# Autodesk Inventor assembly: zlozenieTymRazemOdwrotniezUchwytem
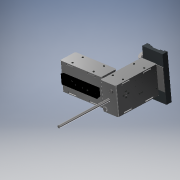
[picture p0: Inventor's stored thumbnail of the model, 180x180]
Saved by Autodesk Inventor 2019.4 (Build 234330000, 330)
## iProperties
Created: 2020-08-29
Part Number: zlozenieTymRazemOdwrotniezUchwytem
Document SubType Name: Assembly
Designer: estee
Author: estee
## Documents named in this file (16)
- F:\GitHub\MUMv2\Equatorial-Mount-MUM\Mechanika\Moduł obrotu RET Estera\projejt\projejt\NoweZlozenie\zlozenieTymRazemOdwrotniezUchwytem.iam
- F:\GitHub\MUMv2\Equatorial-Mount-MUM\Mechanika\Moduł obrotu RET Estera\projejt\projejt\NoweZlozenie\ObudowaNowa.iam
- F:\GitHub\MUMv2\Equatorial-Mount-MUM\Mechanika\Moduł obrotu RET Estera\projejt\projejt\NoweZlozenie\ObudowaNowa2.iam
- F:\GitHub\MUMv2\Equatorial-Mount-MUM\Mechanika\Moduł obrotu RET Estera\projejt\projejt\NoweZlozenie\ISO 4026 - M3 x 3 - ISO.ipt
- F:\GitHub\MUMv2\Equatorial-Mount-MUM\Mechanika\Moduł obrotu RET Estera\projejt\projejt\NoweZlozenie\trzymak.iam
- F:\GitHub\MUMv2\Equatorial-Mount-MUM\Mechanika\Moduł obrotu RET Estera\projejt\projejt\NoweZlozenie\dovetail.ipt
- F:\GitHub\MUMv2\Equatorial-Mount-MUM\Mechanika\Moduł obrotu RET Estera\projejt\projejt\NoweZlozenie\Połączenie gwintowe1.iam
- F:\GitHub\MUMv2\Equatorial-Mount-MUM\Mechanika\Moduł obrotu RET Estera\projejt\projejt\NoweZlozenie\Połączenie gwintowe2.iam
- F:\GitHub\MUMv2\Equatorial-Mount-MUM\Mechanika\Moduł obrotu RET Estera\projejt\projejt\NoweZlozenie\Połączenie gwintowe4.iam
- F:\GitHub\MUMv2\Equatorial-Mount-MUM\Mechanika\Moduł obrotu RET Estera\projejt\projejt\NoweZlozenie\Połączenie gwintowe5.iam
- F:\GitHub\MUMv2\Equatorial-Mount-MUM\Mechanika\Moduł obrotu RET Estera\projejt\projejt\NoweZlozenie\Połączenie gwintowe6.iam
- F:\GitHub\MUMv2\Equatorial-Mount-MUM\Mechanika\Moduł obrotu RET Estera\projejt\projejt\NoweZlozenie\Połączenie gwintowe7.iam
- F:\GitHub\MUMv2\Equatorial-Mount-MUM\Mechanika\Moduł obrotu RET Estera\projejt\projejt\NoweZlozenie\Połączenie gwintowe8.iam
- F:\GitHub\MUMv2\Equatorial-Mount-MUM\Mechanika\Moduł obrotu RET Estera\projejt\projejt\NoweZlozenie\Połączenie gwintowe9.iam
- F:\GitHub\MUMv2\Equatorial-Mount-MUM\Mechanika\Moduł obrotu RET Estera\projejt\projejt\NoweZlozenie\ISO 8676 - M10 x 1 x 20 - ISO.ipt
- F:\GitHub\MUMv2\Equatorial-Mount-MUM\Mechanika\Moduł obrotu RET Estera\projejt\projejt\NoweZlozenie\ISO 4035 - M10 - ISO.ipt
## Components (34 placed, 8 different names)
1. ObudowaNowa:1 [sub-assembly] — Angle:1, Tangent:1, Tangent:2, Tangent:3, Tangent:4, Mate:14, Mate:15, Zestawiające:16, Zestawiające:17, Zestawiające:18, Mate:35, Mate:36, Mate:38, Mate:39, Mate:40, Mate:42, Mate:43, Mate:44, Mate:45, Mate:46, Mate:47, Mate:48, Mate:49, Mate:50
2. ObudowaNowa2:1 [sub-assembly] — Angle:1, Mate:3, Mate:4, Mate:5, Mate:6, Mate:7, Mate:8, Angle:2, Tangent:5, Tangent:6, Mate:13, Mate:14, Mate:15, Mate:51, Mate:52, Mate:53, Mate:54, Mate:55, Mate:56, Mate:57, Mate:58, Mate:59, Mate:60, Mate:61, Mate:62, Mate:63, Mate:64, Mate:65, Mate:66
3. ISO 4026 M3 x 3:1 — Mate:7, Tangent:4
4. ISO 4026 M3 x 3:2 — Mate:5, Tangent:3
5. ISO 4026 M3 x 3:3 — Mate:3, Mate:6, Tangent:1
6. ISO 4026 M3 x 3:4 — Mate:4, Tangent:2
7. trzymak:1 [sub-assembly] — Mate:8, Angle:2, Mate:11, Mate:12, Mate:13
8. ISO 4026 M3 x 3:5 — Mate:11, Tangent:5
9. ISO 4026 M3 x 3:6 — Mate:12, Tangent:6
10. dovetail:1 — Zestawiające:16, Zestawiające:17, Zestawiające:18, Zestawiające:19, Zestawiające:20, Zestawiające:21, Zestawiające:22, Zestawiające:23, Zestawiające:24, Zestawiające:25, Zestawiające:26, Zestawiające:27, Zestawiające:28, Zestawiające:29, Zestawiające:30, Zestawiające:31, Zestawiające:32, Zestawiające:33, Zestawiające:34
11. Połączenie gwintowe:1 [sub-assembly] — Zestawiające:19, Zestawiające:20
12. Połączenie gwintowe:2 [sub-assembly] — Zestawiające:21, Zestawiające:22
13. Połączenie gwintowe:3 [sub-assembly] — Zestawiające:23, Zestawiające:24
14. Połączenie gwintowe:4 [sub-assembly] — Zestawiające:25, Zestawiające:26
15. Połączenie gwintowe:5 [sub-assembly] — Zestawiające:27, Zestawiające:28
16. Połączenie gwintowe:6 [sub-assembly] — Zestawiające:29, Zestawiające:30
17. Połączenie gwintowe:7 [sub-assembly] — Zestawiające:31, Zestawiające:32
18. Połączenie gwintowe:8 [sub-assembly] — Zestawiające:33, Zestawiające:34
19. ISO 8676 M10 x 1 x 20:1 — Mate:35, Mate:36, Mate:37
20. ISO 4035 M10:1 — Mate:37, Mate:38
21. ISO 8676 M10 x 1 x 20:2 — Mate:39, Mate:40, Mate:41
22. ISO 4035 M10:2 — Mate:41, Mate:42
23. ISO 4035 M10:3 — Mate:43, Mate:44
24. ISO 4035 M10:4 — Mate:45, Mate:46
25. ISO 8676 M10 x 1 x 20:3 — Mate:47, Mate:49
26. ISO 8676 M10 x 1 x 20:4 — Mate:48, Mate:50
27. ISO 4035 M10:5 — Mate:51, Mate:54
28. ISO 4035 M10:6 — Mate:55, Mate:56
29. ISO 4035 M10:7 — Mate:52, Mate:53
30. ISO 4035 M10:8 — Mate:57, Mate:58
31. ISO 8676 M10 x 1 x 20:5 — Mate:59, Mate:61
32. ISO 8676 M10 x 1 x 20:6 — Mate:60, Mate:62
33. ISO 8676 M10 x 1 x 20:7 — Mate:65, Mate:66
34. ISO 8676 M10 x 1 x 20:8 — Mate:63, Mate:64
## Relationships (70: Mate 62, Tangent 6, Angle 2)
- Angle:1 (0 deg): ObudowaNowa:1 ↔ ObudowaNowa2:1
- Mate:3: ObudowaNowa2:1 ↔ ISO 4026 M3 x 3:3
- Mate:4: ObudowaNowa2:1 ↔ ISO 4026 M3 x 3:4
- Mate:5: ObudowaNowa2:1 ↔ ISO 4026 M3 x 3:2
- Mate:6: ObudowaNowa2:1 ↔ ISO 4026 M3 x 3:3
- Tangent:1: ObudowaNowa:1 ↔ ISO 4026 M3 x 3:3
- Tangent:2: ObudowaNowa:1 ↔ ISO 4026 M3 x 3:4
- Tangent:3: ObudowaNowa:1 ↔ ISO 4026 M3 x 3:2
- Mate:7: ObudowaNowa2:1 ↔ ISO 4026 M3 x 3:1
- Tangent:4: ObudowaNowa:1 ↔ ISO 4026 M3 x 3:1
- Mate:8: ObudowaNowa2:1 ↔ trzymak:1
- Angle:2 (0 deg): ObudowaNowa2:1 ↔ trzymak:1
- Mate:11: trzymak:1 ↔ ISO 4026 M3 x 3:5
- Tangent:5: ObudowaNowa2:1 ↔ ISO 4026 M3 x 3:5
- Mate:12: trzymak:1 ↔ ISO 4026 M3 x 3:6
- Tangent:6: ObudowaNowa2:1 ↔ ISO 4026 M3 x 3:6
- Mate:13: ObudowaNowa2:1 ↔ trzymak:1
- Mate:14: ObudowaNowa:1 ↔ ObudowaNowa2:1
- Mate:15 (5 mm): ObudowaNowa:1 ↔ ObudowaNowa2:1
- Zestawiające:16 [Mate]: ObudowaNowa:1 ↔ dovetail:1
- Zestawiające:17 [Mate]: ObudowaNowa:1 ↔ dovetail:1
- Zestawiające:18 [Mate]: ObudowaNowa:1 ↔ dovetail:1
- Zestawiające:19 [Mate]: dovetail:1 ↔ Połączenie gwintowe:1
- Zestawiające:20 [Mate]: dovetail:1 ↔ Połączenie gwintowe:1
- Zestawiające:21 [Mate]: dovetail:1 ↔ Połączenie gwintowe:2
- Zestawiające:22 [Mate]: dovetail:1 ↔ Połączenie gwintowe:2
- Zestawiające:23 [Mate]: dovetail:1 ↔ Połączenie gwintowe:3
- Zestawiające:24 [Mate]: dovetail:1 ↔ Połączenie gwintowe:3
- Zestawiające:25 [Mate]: dovetail:1 ↔ Połączenie gwintowe:4
- Zestawiające:26 [Mate]: dovetail:1 ↔ Połączenie gwintowe:4
- Zestawiające:27 [Mate]: dovetail:1 ↔ Połączenie gwintowe:5
- Zestawiające:28 [Mate]: dovetail:1 ↔ Połączenie gwintowe:5
- Zestawiające:29 [Mate]: dovetail:1 ↔ Połączenie gwintowe:6
- Zestawiające:30 [Mate]: dovetail:1 ↔ Połączenie gwintowe:6
- Zestawiające:31 [Mate]: dovetail:1 ↔ Połączenie gwintowe:7
- Zestawiające:32 [Mate]: dovetail:1 ↔ Połączenie gwintowe:7
- Zestawiające:33 [Mate]: dovetail:1 ↔ Połączenie gwintowe:8
- Zestawiające:34 [Mate]: dovetail:1 ↔ Połączenie gwintowe:8
- Mate:35: ObudowaNowa:1 ↔ ISO 8676 M10 x 1 x 20:1
- Mate:36: ObudowaNowa:1 ↔ ISO 8676 M10 x 1 x 20:1
- Mate:37: ISO 8676 M10 x 1 x 20:1 ↔ ISO 4035 M10:1
- Mate:38: ObudowaNowa:1 ↔ ISO 4035 M10:1
- Mate:39: ObudowaNowa:1 ↔ ISO 8676 M10 x 1 x 20:2
- Mate:40: ObudowaNowa:1 ↔ ISO 8676 M10 x 1 x 20:2
- Mate:41: ISO 8676 M10 x 1 x 20:2 ↔ ISO 4035 M10:2
- Mate:42: ObudowaNowa:1 ↔ ISO 4035 M10:2
- Mate:43: ObudowaNowa:1 ↔ ISO 4035 M10:3
- Mate:44: ObudowaNowa:1 ↔ ISO 4035 M10:3
- Mate:45: ObudowaNowa:1 ↔ ISO 4035 M10:4
- Mate:46: ObudowaNowa:1 ↔ ISO 4035 M10:4
- Mate:47: ObudowaNowa:1 ↔ ISO 8676 M10 x 1 x 20:3
- Mate:48: ObudowaNowa:1 ↔ ISO 8676 M10 x 1 x 20:4
- Mate:49: ObudowaNowa:1 ↔ ISO 8676 M10 x 1 x 20:3
- Mate:50: ObudowaNowa:1 ↔ ISO 8676 M10 x 1 x 20:4
- Mate:51: ObudowaNowa2:1 ↔ ISO 4035 M10:5
- Mate:52: ObudowaNowa2:1 ↔ ISO 4035 M10:7
- Mate:53: ObudowaNowa2:1 ↔ ISO 4035 M10:7
- Mate:54: ObudowaNowa2:1 ↔ ISO 4035 M10:5
- Mate:55: ObudowaNowa2:1 ↔ ISO 4035 M10:6
- Mate:56: ObudowaNowa2:1 ↔ ISO 4035 M10:6
- Mate:57: ObudowaNowa2:1 ↔ ISO 4035 M10:8
- Mate:58: ObudowaNowa2:1 ↔ ISO 4035 M10:8
- Mate:59: ObudowaNowa2:1 ↔ ISO 8676 M10 x 1 x 20:5
- Mate:60: ObudowaNowa2:1 ↔ ISO 8676 M10 x 1 x 20:6
- Mate:61: ObudowaNowa2:1 ↔ ISO 8676 M10 x 1 x 20:5
- Mate:62: ObudowaNowa2:1 ↔ ISO 8676 M10 x 1 x 20:6
- Mate:63: ObudowaNowa2:1 ↔ ISO 8676 M10 x 1 x 20:8
- Mate:64: ObudowaNowa2:1 ↔ ISO 8676 M10 x 1 x 20:8
- Mate:65: ObudowaNowa2:1 ↔ ISO 8676 M10 x 1 x 20:7
- Mate:66: ObudowaNowa2:1 ↔ ISO 8676 M10 x 1 x 20:7
